# Autodesk Inventor assembly: CollectorPrototype
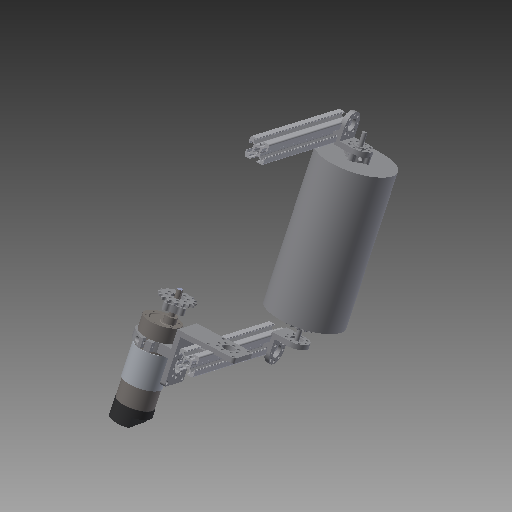
[picture p0: Inventor's stored thumbnail of the model, 512x512]
Saved by Autodesk Inventor 2017 (Build 210142000, 142)
## iProperties
Created: 2016-12-07
Part Number: CollectorPrototype
Document SubType Name: Assembly
Designer: Delta
Author: Delta
## Documents named in this file (12)
- C:\Robotics\CAD\2016-17_CAD\CollectorPrototype.iam
- C:\Robotics\CAD\2016-17_CAD\8InchAx.ipt
- C:\Robotics\CAD\2016-17_CAD\CollectorBrush.ipt
- C:\Robotics\CAD\COTSParts\Actobotics\615 parts\615102.ipt
- C:\Robotics\CAD\COTSParts\Actobotics\545 parts\545400.ipt
- C:\Robotics\CAD\COTSParts\Actobotics\545 parts\545576.ipt
- C:\Robotics\CAD\COTSParts\Actobotics\585 parts\585494.ipt
- C:\Robotics\CAD\COTSParts\Actobotics\am-3102NeveRest20 (1).ipt
- C:\Robotics\CAD\COTSParts\Actobotics\555 parts\555116.ipt
- C:\Robotics\CAD\COTSParts\Actobotics\535 parts\535216.ipt
- C:\Robotics\CAD\COTSParts\Bosch Extrusion\6mm block nut M4.ipt
- C:\Robotics\CAD\COTSParts\Bosch Extrusion\Bosch 20x20 6 in.ipt
## Components (22 placed, 11 different names)
1. 8InchAx:1 — Insert:7, Mate:51
2. CollectorBrush:1 — Insert:12, Insert:13
3. 615102:1 — Insert:10, Insert:11
4. 545400:1 — Mate:5, Mate:8, Mate:11, Mate:12, Mate:13, Mate:14
5. 545400:2 — Mate:6, Mate:7, Mate:31, Mate:33, Insert:10, Insert:14, Insert:15
6. 545576:1 — Insert:11, Insert:12
7. 545576:2 — Mate:39
8. 585494:1 — Mate:9, Mate:10, Insert:27, Mate:27, Mate:28, Mate:29
9. 615102:2 — Mate:39, Insert:28
10. am-3102NeveRest20 (1):1 — Insert:9, Insert:28
11. 555116:1 — Mate:9, Mate:10, Mate:29, Insert:9
12. 535216:1 — Mate:5, Mate:8, Mate:51
13. 535216:2 — Mate:6, Mate:7, Insert:7
14. 6mm block nut M4:1 — Mate:31, Mate:42, Flush:1, Insert:15
15. 6mm block nut M4:2 — Mate:27, Mate:28, Mate:53, Flush:3
16. 6mm block nut M4:3 — Mate:11, Mate:12, Mate:46, Mate:47
17. 6mm block nut M4:4 — Mate:13, Mate:14, Mate:45, Mate:48, Flush:2
18. 6mm block nut M4:5 — Insert:27, Mate:50, Mate:52
19. 6mm block nut M4:6 — Mate:33, Mate:41, Mate:43, Mate:44, Insert:14
20. Bosch 20x20 6 in:1 — Mate:42, Mate:43, Mate:44, Flush:1, Mate:49, Mate:50, Mate:52, Mate:53, Flush:3
21. Bosch 20x20 6 in:2 — Mate:41, Mate:45, Mate:46, Mate:47, Mate:48, Flush:2, Mate:49
22. 545576:3 — Insert:13
## Relationships (42: Mate 29, Insert 10, Flush 3)
- Mate:5: 545400:1 ↔ 535216:1
- Mate:6: 545400:2 ↔ 535216:2
- Mate:7: 545400:2 ↔ 535216:2
- Insert:7: 8InchAx:1 ↔ 535216:2
- Mate:8: 545400:1 ↔ 535216:1
- Mate:9: 585494:1 ↔ 555116:1
- Mate:10: 585494:1 ↔ 555116:1
- Mate:11: 545400:1 ↔ 6mm block nut M4:3
- Mate:12: 545400:1 ↔ 6mm block nut M4:3
- Mate:13: 545400:1 ↔ 6mm block nut M4:4
- Mate:14: 545400:1 ↔ 6mm block nut M4:4
- Insert:27: 585494:1 ↔ 6mm block nut M4:5
- Mate:27: 585494:1 ↔ 6mm block nut M4:2
- Mate:28: 585494:1 ↔ 6mm block nut M4:2
- Mate:29: 585494:1 ↔ 555116:1
- Mate:31: 545400:2 ↔ 6mm block nut M4:1
- Mate:33: 545400:2 ↔ 6mm block nut M4:6
- Insert:9: am-3102NeveRest20 (1):1 ↔ 555116:1
- Mate:39: 545576:2 ↔ 615102:2
- Mate:41: 6mm block nut M4:6 ↔ Bosch 20x20 6 in:2
- Mate:42: 6mm block nut M4:1 ↔ Bosch 20x20 6 in:1
- Mate:43: 6mm block nut M4:6 ↔ Bosch 20x20 6 in:1
- Mate:44: 6mm block nut M4:6 ↔ Bosch 20x20 6 in:1
- Flush:1: 6mm block nut M4:1 ↔ Bosch 20x20 6 in:1
- Mate:45: 6mm block nut M4:4 ↔ Bosch 20x20 6 in:2
- Mate:46: 6mm block nut M4:3 ↔ Bosch 20x20 6 in:2
- Mate:47: 6mm block nut M4:3 ↔ Bosch 20x20 6 in:2
- Mate:48: 6mm block nut M4:4 ↔ Bosch 20x20 6 in:2
- Flush:2: 6mm block nut M4:4 ↔ Bosch 20x20 6 in:2
- Insert:10 (13.97 mm): 615102:1 ↔ 545400:2
- Insert:11: 615102:1 ↔ 545576:1
- Insert:12: CollectorBrush:1 ↔ 545576:1
- Mate:49 (186.817 mm): Bosch 20x20 6 in:1 ↔ Bosch 20x20 6 in:2
- Insert:13: CollectorBrush:1 ↔ 545576:3
- Insert:14: 545400:2 ↔ 6mm block nut M4:6
- Insert:15: 545400:2 ↔ 6mm block nut M4:1
- Mate:50: 6mm block nut M4:5 ↔ Bosch 20x20 6 in:1
- Mate:51: 8InchAx:1 ↔ 535216:1
- Mate:52: 6mm block nut M4:5 ↔ Bosch 20x20 6 in:1
- Mate:53: 6mm block nut M4:2 ↔ Bosch 20x20 6 in:1
- Flush:3 (23.368 mm): 6mm block nut M4:2 ↔ Bosch 20x20 6 in:1
- Insert:28 (7.4422 mm): 615102:2 ↔ am-3102NeveRest20 (1):1
